# Autodesk Inventor assembly: ramp
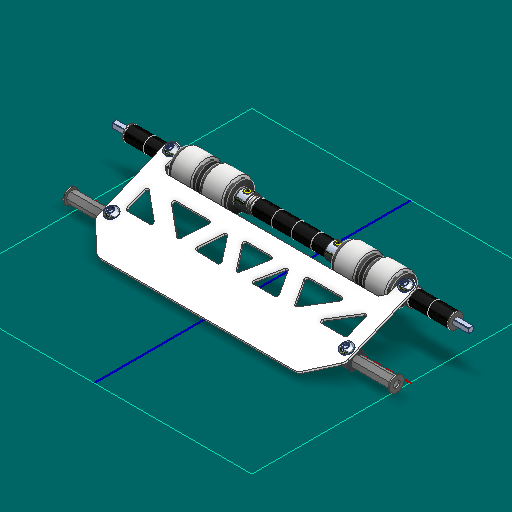
[picture p0: Inventor's stored thumbnail of the model, 512x512]
Saved by Autodesk Inventor 2025 (Build 290162000, 162)
## iProperties
Created: 2024-08-22
Part Number: ramp
Document SubType Name: Assembly
Designer: averey
Author: averey
## Documents named in this file (10)
- C:\Users\avere\vex_robotics_high_stakes\hardware\cad\bots\ENIGMA\intake\first_stage\ramp.iam
- C:\Users\avere\vex_robotics_high_stakes\hardware\cad\bots\ENIGMA\intake\first_stage\bottom_roller.iam
- C:\Users\avere\vex_robotics_high_stakes\hardware\cad\VEX-CAD-Inventor\Structure\Standoff\Standoff 1.00.ipt
- C:\Users\avere\vex_robotics_high_stakes\hardware\cad\VEX-CAD-Inventor\Structure\Standoff.ipt
- C:\Users\avere\vex_robotics_high_stakes\hardware\cad\VEX-CAD-Inventor\Motion\Shaft LS\Shaft Collar ipts\Shaft Collar No Screw.ipt
- C:\Users\avere\vex_robotics_high_stakes\hardware\cad\VEX-CAD-Inventor\Motion\Spacers\Washer Steel.ipt
- C:\Users\avere\vex_robotics_high_stakes\hardware\cad\VEX-CAD-Inventor\Motion\Spacers\Washer Steel\SWasher .375 OD x .031250.ipt
- C:\Users\avere\vex_robotics_high_stakes\hardware\cad\bots\ENIGMA\intake\first_stage\custom_parts\ramp.ipt
- C:\Users\avere\vex_robotics_high_stakes\hardware\cad\VEX-CAD-Inventor\Structure\Hardware\Screw Steel - Star\SScrew Star Smooth .250.ipt
- C:\Users\avere\vex_robotics_high_stakes\hardware\cad\VEX-CAD-Inventor\Structure\Hardware\Screw Steel - Star.ipt
## Components (12 placed, 6 different names)
1. bottom_roller:1 [sub-assembly] — Insert:9, Mate:1
2. Standoff 1.00:1
3. Shaft Collar No Screw:1 — Mate:2, Insert:10
4. Standoff 1.00:2 — Insert:8
5. Shaft Collar No Screw:2 — Mate:2, Mate:3
6. SWasher .375 OD x .031250:2
7. ramp:1 — Insert:9, Mate:1, Mate:3, Insert:10, Insert:11, Insert:12, Insert:13, Insert:14
8. SWasher .375 OD x .031250:3 — Insert:8
9. SScrew Star Smooth .250:1 — Insert:11
10. SScrew Star Smooth .250:2 — Insert:12
11. SScrew Star Smooth .250:3 — Insert:14
12. SScrew Star Smooth .250:4 — Insert:13
## Relationships (13: Insert 10, Mate 3)
- [Insert]: Standoff 1.00:1 ↔ Shaft Collar No Screw:1
- [Insert]: Standoff 1.00:2 ↔ Shaft Collar No Screw:2
- [Insert]: Standoff 1.00:1 ↔ SWasher .375 OD x .031250:2
- Insert:8: Standoff 1.00:2 ↔ SWasher .375 OD x .031250:3
- Insert:9: bottom_roller:1 ↔ ramp:1
- Mate:1: bottom_roller:1 ↔ ramp:1
- Mate:2: Shaft Collar No Screw:1 ↔ Shaft Collar No Screw:2
- Mate:3: Shaft Collar No Screw:2 ↔ ramp:1
- Insert:10: Shaft Collar No Screw:1 ↔ ramp:1
- Insert:11: ramp:1 ↔ SScrew Star Smooth .250:1
- Insert:12: ramp:1 ↔ SScrew Star Smooth .250:2
- Insert:13: ramp:1 ↔ SScrew Star Smooth .250:4
- Insert:14: ramp:1 ↔ SScrew Star Smooth .250:3
## Named parameters: d31_d30 = 0 mm
